# Autodesk Inventor assembly: IM_Matchboxscope_plate_3 MB bg
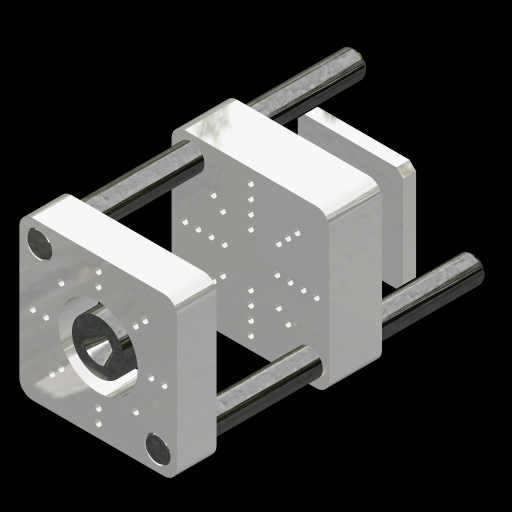
[picture p0: Inventor's stored thumbnail of the model, 512x512]
Saved by Autodesk Inventor 2024 (Build 280153000, 153)
## iProperties
Created: 2023-06-29
Part Number: IM_Matchboxscope_plate_3 MB bg
Document SubType Name: Assembly
Designer: buchmannmartin
Author: buchmannmartin
## Documents named in this file (3)
- E:\User\Dokumente\#BeneEspressoscope\IM_Matchboxscope_plate_3 MB bg.iam
- E:\User\Dokumente\#BeneEspressoscope\MicroPlast-MB-BG.iam
- E:\User\Dokumente\#BeneEspressoscope\IM_Matchboxscope_plate_3 MB Layout.ipt
## Components (2 placed, 2 different names)
1. MicroPlast-MB-BG:1 [sub-assembly] — Passend:1, Passend:2
2. IM_Matchboxscope_plate_3 MB Layout:1 — Passend:1, Fluchtend:1, Passend:2
## Relationships (3: Mate 2, Flush 1)
- Passend:1 [Mate]: MicroPlast-MB-BG:1 ↔ IM_Matchboxscope_plate_3 MB Layout:1
- Fluchtend:1 [Flush]: IM_Matchboxscope_plate_3 MB Layout:1
- Passend:2 [Mate]: MicroPlast-MB-BG:1 ↔ IM_Matchboxscope_plate_3 MB Layout:1
